# Autodesk Inventor assembly: FullAssem
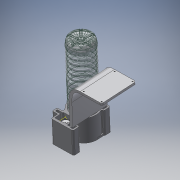
[picture p0: Inventor's stored thumbnail of the model, 180x180]
Saved by Autodesk Inventor 2019 (Build 230136000, 136)
## iProperties
Created: 2019-04-09
Part Number: FullAssem
Document SubType Name: Assembly
Designer: Jorian Brusind
Author: Jorian Brusind
## Documents named in this file (5)
- C:\Users\Jorian Bruslind\Documents\GitHub\PersonalProjects\Automated Terrarium Project\Inventor Files\V3\FullAssem.iam
- C:\Users\Jorian Bruslind\Documents\GitHub\PersonalProjects\Automated Terrarium Project\Inventor Files\V3\mini_pump.ipt
- C:\Users\Jorian Bruslind\Documents\GitHub\PersonalProjects\Automated Terrarium Project\Inventor Files\V3\Bottle 600ml.iam
- C:\Users\Jorian Bruslind\Documents\GitHub\PersonalProjects\Automated Terrarium Project\Inventor Files\V3\BoitCase.ipt
- C:\Users\Jorian Bruslind\Documents\GitHub\PersonalProjects\Automated Terrarium Project\Inventor Files\V3\Backplate.ipt
## Components (4 placed, 4 different names)
1. Bottle 600ml:1 [sub-assembly] — Mate:2
2. BoitCase:1 — Mate:2, Mate:4, Mate:6, Mate:7
3. mini_pump:1 — Mate:7
4. Backplate:1 — Mate:4, Mate:6
## Relationships (4: Mate 4)
- Mate:2: Bottle 600ml:1 ↔ BoitCase:1
- Mate:4: BoitCase:1 ↔ Backplate:1
- Mate:6: BoitCase:1 ↔ Backplate:1
- Mate:7: BoitCase:1 ↔ mini_pump:1
